# Autodesk Inventor assembly: Shelf
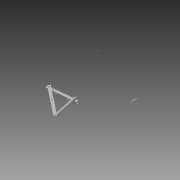
[picture p0: Inventor's stored thumbnail of the model, 180x180]
Saved by Autodesk Inventor 2013 (Build 170138000, 138)
## iProperties
Created: 2014-05-22
Part Number: Shelf
Document SubType Name: Assembly
Designer: nojessen
Mass: 1766.78 g
Surface Area: 1327.56 cm^2
Volume: 225.068 cm^3
Density: 7.85 g/cm^3
Author: nojessen
## Documents named in this file (7)
- C:\Users\nojessen\Documents\GitHub\IED_Virtual_Design_Challenge\CAD\Shelf.iam
- C:\Users\nojessen\Documents\GitHub\IED_Virtual_Design_Challenge\CAD\Clip for Pin.ipt
- C:\Users\nojessen\Documents\GitHub\IED_Virtual_Design_Challenge\CAD\Horizantal Rod.ipt
- C:\Users\nojessen\Documents\GitHub\IED_Virtual_Design_Challenge\CAD\Pin.ipt
- C:\Users\nojessen\Documents\GitHub\IED_Virtual_Design_Challenge\CAD\Vertical Rod.ipt
- C:\Users\nojessen\Documents\GitHub\IED_Virtual_Design_Challenge\CAD\Piece One-Diagonal Piece.ipt
- C:\Users\nojessen\Documents\GitHub\IED_Virtual_Design_Challenge\CAD\Piece Two-Diagonal Piece.ipt
## Components (8 placed, 6 different names)
1. Clip for Pin:1
2. Horizantal Rod:1 — Mate:1, Mate:2, Mate:3
3. Vertical Rod:1 — Mate:1, Mate:2, Mate:4, Mate:5
4. Pin:1 — Mate:8, Mate:9
5. Pin:2
6. Pin:3 — Mate:10, Mate:11
7. Piece One-Diagonal Piece:1 — Mate:3, Mate:6, Mate:7, Flush:1, Mate:8, Mate:9
8. Piece Two-Diagonal Piece:1 — Mate:4, Mate:5, Mate:6, Mate:7, Flush:1, Mate:10, Mate:11
## Relationships (12: Mate 11, Flush 1)
- Mate:1: Horizantal Rod:1 ↔ Vertical Rod:1
- Mate:2 (12.7 mm): Horizantal Rod:1 ↔ Vertical Rod:1
- Mate:3: Horizantal Rod:1 ↔ Piece One-Diagonal Piece:1
- Mate:4: Vertical Rod:1 ↔ Piece Two-Diagonal Piece:1
- Mate:5: Vertical Rod:1 ↔ Piece Two-Diagonal Piece:1
- Mate:6: Piece One-Diagonal Piece:1 ↔ Piece Two-Diagonal Piece:1
- Mate:7: Piece One-Diagonal Piece:1 ↔ Piece Two-Diagonal Piece:1
- Flush:1: Piece One-Diagonal Piece:1 ↔ Piece Two-Diagonal Piece:1
- Mate:8: Pin:1 ↔ Piece One-Diagonal Piece:1
- Mate:9: Pin:1 ↔ Piece One-Diagonal Piece:1
- Mate:10: Pin:3 ↔ Piece Two-Diagonal Piece:1
- Mate:11: Pin:3 ↔ Piece Two-Diagonal Piece:1
